# Autodesk Inventor assembly: endmould_top_v3_p1
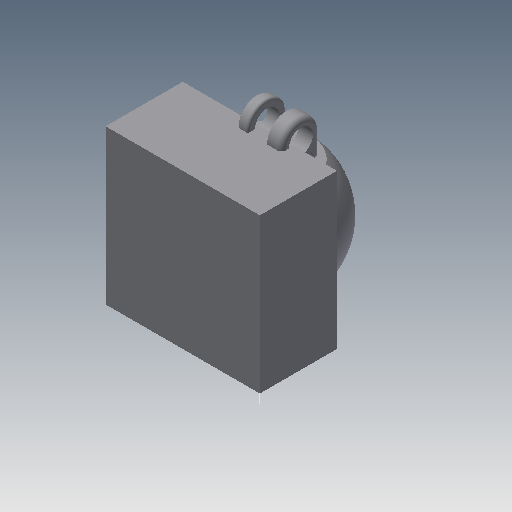
[picture p0: Inventor's stored thumbnail of the model, 512x512]
Saved by Autodesk Inventor 2017 (Build 210142000, 142)
## iProperties
Created: 2018-07-06
Part Number: endmould_top_v3_p1
Document SubType Name: Assembly
Designer: Nic
Author: Nic
## Documents named in this file (4)
- C:\Users\Nic\Documents\Antenna\endmould_top_v3_p1.iam
- C:\Users\Nic\Documents\Antenna\mould_casing.ipt
- C:\Users\Nic\Documents\Antenna\end_segment_v3.ipt
- C:\Users\Nic\Documents\Antenna\end_pad.ipt
## Components (3 placed, 3 different names)
1. mould_casing:1 — Insert:1, Ball:1, Angle:1
2. end_segment_v3:1 — Insert:1
3. end_pad:1 — Ball:1, Angle:1
## Relationships (3: Insert 1, BallJoint 1, Angle 1)
- Insert:1: mould_casing:1 ↔ end_segment_v3:1
- Ball:1: mould_casing:1 ↔ end_pad:1
- Angle:1 (0 deg): mould_casing:1 ↔ end_pad:1
